# Autodesk Inventor assembly: rail_MIR
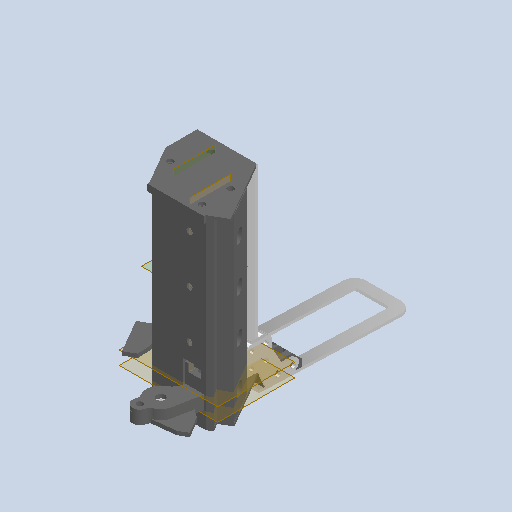
[picture p0: Inventor's stored thumbnail of the model, 512x512]
Saved by Autodesk Inventor 2024.1 (Build 281209000, 209)
## iProperties
Created: 2025-01-17
Part Number: rail_MIR
Document SubType Name: Assembly
Designer: hibik
Author: hibik
## Documents named in this file (11)
- C:\Users\hibik\Documents\Robomech\RESCUE\ORCA\hard\fork\right\rail_MIR.iam
- C:\Users\hibik\Documents\Robomech\RESCUE\ORCA\hard\fork\right\rail_base_MIR.ipt
- C:\Users\hibik\Documents\Robomech\RESCUE\ORCA\hard\fork\right\rail_rail_MIR.ipt
- C:\Users\hibik\Documents\Robomech\RESCUE\ORCA\hard\fork\right\rail_cover_upper_MIR.ipt
- C:\Users\hibik\Documents\Robomech\RESCUE\ORCA\hard\fork\right\rail_cover_under_MIR.ipt
- C:\Users\hibik\Documents\Robomech\RESCUE\ORCA\hard\fork\right\rail_roller_MIR.ipt
- C:\Users\hibik\Documents\Robomech\RESCUE\ORCA\hard\fork\right\fork_MIR.iam
- C:\Users\hibik\Documents\Robomech\RESCUE\ORCA\hard\fork\right\chain_MIR.iam
- C:\Users\hibik\Documents\Robomech\RESCUE\ORCA\hard\std_parts\screw_M3_MIR.ipt
- C:\Users\hibik\Documents\Robomech\RESCUE\ORCA\hard\fork\right\screw_lift_MIR.iam
- C:\Users\hibik\Documents\Robomech\RESCUE\ORCA\hard\fork\right\rail_backcover_MIR.ipt
## Components (15 placed, 10 different names)
1. rail_base_MIR:1 — フラッシュ:2, フラッシュ:1, メイト:1, フラッシュ:8, フラッシュ:7, 挿入:1, メイト:7, メイト:6, メイト:10, メイト:9, メイト:8, メイト:13, メイト:11
2. rail_rail_MIR:1 — フラッシュ:2, フラッシュ:1, メイト:1, メイト:2, メイト:3, フラッシュ:6, フラッシュ:5, 正接:2, 正接:1, メイト:4, 挿入:2, 挿入:3, 挿入:4, 挿入:5, 挿入:6, 挿入:7
3. rail_cover_upper_MIR:1 — フラッシュ:8, フラッシュ:7, メイト:2, メイト:5, メイト:12
4. rail_cover_under_MIR:1 — メイト:3, フラッシュ:6, フラッシュ:5
5. rail_roller_MIR:1 — 挿入:1
6. fork_MIR:1 [sub-assembly] — 正接:2, 正接:1, メイト:4
7. chain_MIR:1 [sub-assembly] — メイト:7, メイト:6, メイト:5
8. screw_M3_MIR:1 — 挿入:2
9. screw_M3_MIR:2 — 挿入:3
10. screw_M3_MIR:3 — 挿入:4
11. screw_M3_MIR:4 — 挿入:5
12. screw_M3_MIR:5 — 挿入:6
13. screw_M3_MIR:6 — 挿入:7
14. screw_lift_MIR:1 [sub-assembly] — メイト:10, メイト:9, メイト:8
15. rail_backcover_MIR:1 — メイト:13, メイト:12, メイト:11
## Relationships (28: Mate 13, Insert 7, Flush 6, Tangent 2)
- フラッシュ:2 [Flush] (-5 mm): rail_base_MIR:1 ↔ rail_rail_MIR:1
- フラッシュ:1 [Flush]: rail_base_MIR:1 ↔ rail_rail_MIR:1
- メイト:1 [Mate]: rail_base_MIR:1 ↔ rail_rail_MIR:1
- フラッシュ:8 [Flush]: rail_base_MIR:1 ↔ rail_cover_upper_MIR:1
- フラッシュ:7 [Flush]: rail_base_MIR:1 ↔ rail_cover_upper_MIR:1
- メイト:2 [Mate]: rail_rail_MIR:1 ↔ rail_cover_upper_MIR:1
- メイト:3 [Mate]: rail_rail_MIR:1 ↔ rail_cover_under_MIR:1
- フラッシュ:6 [Flush]: rail_rail_MIR:1 ↔ rail_cover_under_MIR:1
- フラッシュ:5 [Flush]: rail_rail_MIR:1 ↔ rail_cover_under_MIR:1
- 挿入:1 [Insert] (0.25 mm): rail_base_MIR:1 ↔ rail_roller_MIR:1
- 正接:2 [Tangent]: rail_rail_MIR:1 ↔ fork_MIR:1
- 正接:1 [Tangent]: rail_rail_MIR:1 ↔ fork_MIR:1
- メイト:4 [Mate]: rail_rail_MIR:1 ↔ fork_MIR:1
- メイト:7 [Mate] (1 mm): rail_base_MIR:1 ↔ chain_MIR:1
- メイト:6 [Mate] (1 mm): rail_base_MIR:1 ↔ chain_MIR:1
- メイト:5 [Mate] (1 mm): rail_cover_upper_MIR:1 ↔ chain_MIR:1
- 挿入:2 [Insert]: rail_rail_MIR:1 ↔ screw_M3_MIR:1
- 挿入:3 [Insert]: rail_rail_MIR:1 ↔ screw_M3_MIR:2
- 挿入:4 [Insert]: rail_rail_MIR:1 ↔ screw_M3_MIR:3
- 挿入:5 [Insert]: rail_rail_MIR:1 ↔ screw_M3_MIR:4
- 挿入:6 [Insert]: rail_rail_MIR:1 ↔ screw_M3_MIR:5
- 挿入:7 [Insert]: rail_rail_MIR:1 ↔ screw_M3_MIR:6
- メイト:10 [Mate] (0.1 mm): rail_base_MIR:1 ↔ screw_lift_MIR:1
- メイト:9 [Mate] (0.1 mm): rail_base_MIR:1 ↔ screw_lift_MIR:1
- メイト:8 [Mate] (0.2 mm): rail_base_MIR:1 ↔ screw_lift_MIR:1
- メイト:13 [Mate]: rail_base_MIR:1 ↔ rail_backcover_MIR:1
- メイト:12 [Mate]: rail_cover_upper_MIR:1 ↔ rail_backcover_MIR:1
- メイト:11 [Mate]: rail_base_MIR:1 ↔ rail_backcover_MIR:1
